# Autodesk Inventor assembly: gripper
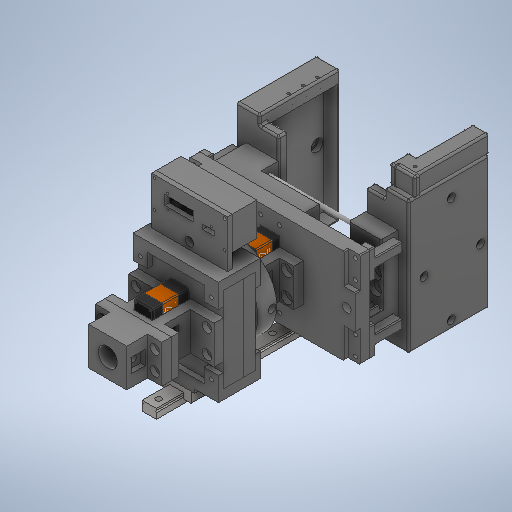
[picture p0: Inventor's stored thumbnail of the model, 512x512]
Saved by Autodesk Inventor 2026.2 (Build 302298010, 298A)
## iProperties
Created: 2026-05-16
Part Number: gripper
Document SubType Name: Assembly
Designer: chris
Author: chris
## Documents named in this file (25)
- C:\Users\chanh\내 드라이브\교과공부\2026년 1학기 (4학년 1학기)\01창의제품설계\CLOSE_hardware\04그리퍼\gripper\gripper.iam
- C:\Users\chanh\내 드라이브\교과공부\2026년 1학기 (4학년 1학기)\01창의제품설계\CLOSE_hardware\04그리퍼\gripper\linear_bracket.ipt
- C:\Users\chanh\내 드라이브\교과공부\2026년 1학기 (4학년 1학기)\01창의제품설계\CLOSE_hardware\04그리퍼\gripper\motor1_bracket.ipt
- C:\Users\chanh\내 드라이브\교과공부\2026년 1학기 (4학년 1학기)\01창의제품설계\CLOSE_hardware\04그리퍼\gripper\rail_top.ipt
- C:\Users\chanh\내 드라이브\교과공부\2026년 1학기 (4학년 1학기)\01창의제품설계\CLOSE_hardware\04그리퍼\gripper\bearing_bracket1.ipt
- C:\Users\chanh\내 드라이브\교과공부\2026년 1학기 (4학년 1학기)\01창의제품설계\CLOSE_hardware\04그리퍼\gripper\bearing_bracket2.ipt
- C:\Users\chanh\내 드라이브\교과공부\2026년 1학기 (4학년 1학기)\01창의제품설계\CLOSE_hardware\04그리퍼\gripper\bearing_bracket3.ipt
- C:\Users\chanh\내 드라이브\교과공부\2026년 1학기 (4학년 1학기)\01창의제품설계\CLOSE_hardware\04그리퍼\gripper\bearing_bracket4.ipt
- C:\Users\chanh\내 드라이브\교과공부\2026년 1학기 (4학년 1학기)\01창의제품설계\CLOSE_hardware\04그리퍼\gripper\motor_bracket3.ipt
- C:\Users\chanh\내 드라이브\교과공부\2026년 1학기 (4학년 1학기)\01창의제품설계\CLOSE_hardware\04그리퍼\gripper\HTD-45H.ipt
- C:\Users\chanh\내 드라이브\교과공부\2026년 1학기 (4학년 1학기)\01창의제품설계\CLOSE_hardware\04그리퍼\gripper\Top Horn.ipt
- C:\Users\chanh\내 드라이브\교과공부\2026년 1학기 (4학년 1학기)\01창의제품설계\CLOSE_hardware\04그리퍼\gripper\MGN15C Cart.ipt
- C:\Users\chanh\내 드라이브\교과공부\2026년 1학기 (4학년 1학기)\01창의제품설계\CLOSE_hardware\04그리퍼\gripper\MGN15 Rail.ipt
- C:\Users\chanh\내 드라이브\교과공부\2026년 1학기 (4학년 1학기)\01창의제품설계\CLOSE_hardware\04그리퍼\gripper\gripper_bracket_finger_right.ipt
- C:\Users\chanh\내 드라이브\교과공부\2026년 1학기 (4학년 1학기)\01창의제품설계\CLOSE_hardware\04그리퍼\gripper\gripper_bracket_finger_left.ipt
- C:\Users\chanh\내 드라이브\교과공부\2026년 1학기 (4학년 1학기)\01창의제품설계\CLOSE_hardware\04그리퍼\gripper\gripper_base - Copy.ipt
- C:\Users\chanh\내 드라이브\교과공부\2026년 1학기 (4학년 1학기)\01창의제품설계\CLOSE_hardware\04그리퍼\gripper\gear2.ipt
- C:\Users\chanh\내 드라이브\교과공부\2026년 1학기 (4학년 1학기)\01창의제품설계\CLOSE_hardware\04그리퍼\gripper\gear1.ipt
- C:\Users\chanh\내 드라이브\교과공부\2026년 1학기 (4학년 1학기)\01창의제품설계\CLOSE_hardware\04그리퍼\gripper\finger2+.ipt
- C:\Users\chanh\내 드라이브\교과공부\2026년 1학기 (4학년 1학기)\01창의제품설계\CLOSE_hardware\04그리퍼\gripper\finger2.ipt
- C:\Users\chanh\내 드라이브\교과공부\2026년 1학기 (4학년 1학기)\01창의제품설계\CLOSE_hardware\04그리퍼\gripper\connecting_part.ipt
- C:\Users\chanh\내 드라이브\교과공부\2026년 1학기 (4학년 1학기)\01창의제품설계\CLOSE_hardware\04그리퍼\gripper\al_rod_bracket_Real.ipt
- C:\Users\chanh\내 드라이브\교과공부\2026년 1학기 (4학년 1학기)\01창의제품설계\CLOSE_hardware\04그리퍼\gripper\al_rod.ipt
- C:\Users\chanh\내 드라이브\교과공부\2026년 1학기 (4학년 1학기)\01창의제품설계\CLOSE_hardware\04그리퍼\gripper\camera\camera_case_new.ipt
- C:\Users\chanh\내 드라이브\교과공부\2026년 1학기 (4학년 1학기)\01창의제품설계\CLOSE_hardware\04그리퍼\gripper\camera\camera_case_new_2.ipt
## Components (33 placed, 24 different names)
1. linear_bracket:1 — Flush:1, Flush:2, Flush:3, Rigid:1
2. motor1_bracket:1 — Rigid:1, Rigid:2, Rigid:3
3. rail_top:1 — Rigid:9, Rigid:10
4. bearing_bracket1:1 — Rigid:3, Rigid:6
5. bearing_bracket2:1 — Rigid:6, Rigid:9, Rigid:25
6. bearing_bracket3:1 — Rigid:4, Rigid:5
7. bearing_bracket4:1 — Rigid:5, Rigid:7, Mate:3
8. motor_bracket3:1 — Mate:2, Mate:3, Mate:4, Rigid:8, Rigid:12
9. HTD-45H:1 — Rigid:2, Rotational:2
10. HTD-45H:2 — Rigid:8, Rotational:1
11. Top Horn:1 — Rotational:2, Rigid:4
12. Top Horn:2 — Rotational:1, Rigid:11
13. MGN15C Cart:1 — Rigid:10, Slider:1
14. MGN15 Rail:1 — Slider:1
15. gripper_bracket_finger_right:1 — Rigid:21, Rigid:23
16. gripper_bracket_finger_left:1 — Rigid:22
17. gripper_base - Copy:1 — Rigid:12, Rigid:13, Rigid:14, Rigid:15, Rigid:16
18. gear2:1 — Mate:5, Mate:6, Mate:7, Rigid:21
19. gear2:2 — Mate:8, Mate:9, Mate:10, Rigid:22
20. gear1:1 — Rigid:11
21. finger2+:1 — Mate:11, Flush:4, Flush:5
22. finger2:1 — Rigid:23, Mate:11, Flush:4, Flush:5
23. connecting_part:1 — Rigid:7, Mate:2, Mate:4
24. al_rod_bracket_Real:1 — Rigid:15, Rigid:19, Rigid:20
25. al_rod_bracket_Real:2 — Rigid:14
26. al_rod_bracket_Real:3 — Rigid:13, Rigid:17, Rigid:18, Mate:10
27. al_rod_bracket_Real:4 — Rigid:16, Mate:7
28. al_rod:1 — Rigid:18, Mate:6
29. al_rod:2 — Rigid:19, Mate:5
30. al_rod:3 — Rigid:20, Mate:9
31. al_rod:4 — Rigid:17, Mate:8
32. camera_case_new:1 — Rigid:24, Rigid:25
33. camera_case_new_2:1 — Rigid:24
## Relationships (43: WeldJoint 25, Mate 10, Flush 5, RevoluteJoint 2, TranslationJoint 1)
- Flush:1: linear_bracket:1
- Flush:2: linear_bracket:1
- Flush:3: linear_bracket:1
- Rigid:1 [WeldJoint]: linear_bracket:1 ↔ motor1_bracket:1
- Rigid:2 [WeldJoint]: motor1_bracket:1 ↔ HTD-45H:1
- Rotational:2 [RevoluteJoint]: HTD-45H:1 ↔ Top Horn:1
- Rigid:3 [WeldJoint]: motor1_bracket:1 ↔ bearing_bracket1:1
- Rigid:4 [WeldJoint]: bearing_bracket3:1 ↔ Top Horn:1
- Rigid:5 [WeldJoint]: bearing_bracket3:1 ↔ bearing_bracket4:1
- Rigid:6 [WeldJoint]: bearing_bracket1:1 ↔ bearing_bracket2:1
- Rigid:7 [WeldJoint]: bearing_bracket4:1 ↔ connecting_part:1
- Mate:2 (0.05 mm): motor_bracket3:1 ↔ connecting_part:1
- Mate:3: bearing_bracket4:1 ↔ motor_bracket3:1
- Mate:4 (0.05 mm): motor_bracket3:1 ↔ connecting_part:1
- Rigid:8 [WeldJoint]: motor_bracket3:1 ↔ HTD-45H:2
- Rotational:1 [RevoluteJoint]: HTD-45H:2 ↔ Top Horn:2
- Rigid:9 [WeldJoint]: rail_top:1 ↔ bearing_bracket2:1
- Rigid:10 [WeldJoint]: rail_top:1 ↔ MGN15C Cart:1
- Slider:1 [TranslationJoint]: MGN15C Cart:1 ↔ MGN15 Rail:1
- Rigid:11 [WeldJoint]: Top Horn:2 ↔ gear1:1
- Rigid:12 [WeldJoint]: motor_bracket3:1 ↔ gripper_base - Copy:1
- Rigid:13 [WeldJoint]: gripper_base - Copy:1 ↔ al_rod_bracket_Real:3
- Rigid:14 [WeldJoint]: gripper_base - Copy:1 ↔ al_rod_bracket_Real:2
- Rigid:15 [WeldJoint]: gripper_base - Copy:1 ↔ al_rod_bracket_Real:1
- Rigid:16 [WeldJoint]: gripper_base - Copy:1 ↔ al_rod_bracket_Real:4
- Rigid:17 [WeldJoint]: al_rod_bracket_Real:3 ↔ al_rod:4
- Rigid:18 [WeldJoint]: al_rod_bracket_Real:3 ↔ al_rod:1
- Rigid:19 [WeldJoint]: al_rod_bracket_Real:1 ↔ al_rod:2
- Rigid:20 [WeldJoint]: al_rod_bracket_Real:1 ↔ al_rod:3
- Mate:5: gear2:1 ↔ al_rod:2
- Mate:6: gear2:1 ↔ al_rod:1
- Mate:7: gear2:1 ↔ al_rod_bracket_Real:4
- Mate:8: gear2:2 ↔ al_rod:4
- Mate:9: gear2:2 ↔ al_rod:3
- Mate:10: gear2:2 ↔ al_rod_bracket_Real:3
- Rigid:21 [WeldJoint]: gripper_bracket_finger_right:1 ↔ gear2:1
- Rigid:22 [WeldJoint]: gripper_bracket_finger_left:1 ↔ gear2:2
- Rigid:23 [WeldJoint]: gripper_bracket_finger_right:1 ↔ finger2:1
- Mate:11: finger2+:1 ↔ finger2:1
- Flush:4: finger2+:1 ↔ finger2:1
- Flush:5: finger2+:1 ↔ finger2:1
- Rigid:24 [WeldJoint]: camera_case_new:1 ↔ camera_case_new_2:1
- Rigid:25 [WeldJoint]: bearing_bracket2:1 ↔ camera_case_new:1
